# Autodesk Inventor assembly: MX-106T_with_Horn_MIR
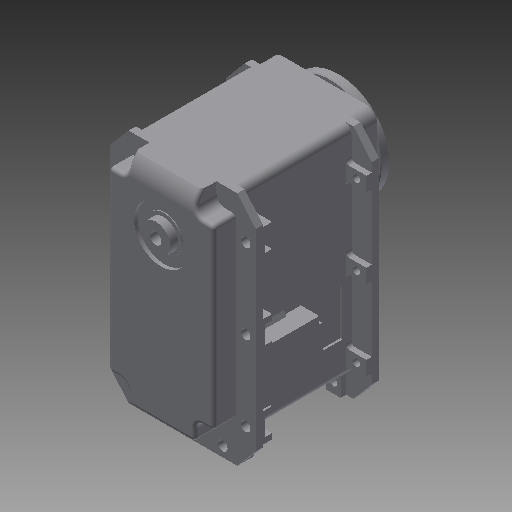
[picture p0: Inventor's stored thumbnail of the model, 512x512]
Saved by Autodesk Inventor 2019 (Build 230136000, 136)
## iProperties
Created: 2015-05-09
Part Number: MX-106T_with_Horn_MIR
Document SubType Name: Assembly
Designer: 4wieser
Author: bitbots
## Documents named in this file (3)
- Z:\Nico_N\NICO-CAD-master\NICO_CAD_master\motors\Mx106\MX-106T_with_Horn_MIR.iam
- Z:\Nico_N\NICO-CAD-master\NICO_CAD_master\motors\Mx106\MX-106T_MIR.ipt
- Z:\Nico_N\NICO-CAD-master\NICO_CAD_master\motors\HN05-N101_(mx64)\HN05-N101_MIR3.ipt
## Components (2 placed, 2 different names)
1. MX-106T_MIR:1 — Rotational:1
2. HN05-N101_MIR3:1 — Rotational:1
## Relationships (1: RevoluteJoint 1)
- Rotational:1 [RevoluteJoint] (-7 mm): MX-106T_MIR:1 ↔ HN05-N101_MIR3:1
